# Autodesk Inventor assembly: GripCharger
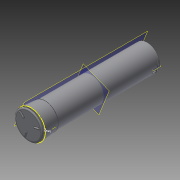
[picture p0: Inventor's stored thumbnail of the model, 180x180]
Saved by Autodesk Inventor 2014 SP1 (Build 180222100, 222)
## iProperties
Created: 2015-10-17
Part Number: GripCharger
Document SubType Name: Assembly
Designer: anthony
Author: anthony
## Documents named in this file (4)
- C:\Users\anthony\Documents\HardwareHack\GripCharger.iam
- C:\Users\anthony\Documents\HardwareHack\GripOuterTube.ipt
- C:\Users\anthony\Documents\HardwareHack\GripScrewCap.ipt
- C:\Users\anthony\Documents\HardwareHack\GripScrewCapCap.ipt
## Components (3 placed, 3 different names)
1. GripOuterTube:1 — Mate:1, Mate:2, Mate:3
2. GripScrewCap:1 — Mate:1, Mate:3
3. GripScrewCapCap:1
## Relationships (3: Mate 3)
- Mate:1: GripOuterTube:1 ↔ GripScrewCap:1
- Mate:2: GripOuterTube:1
- Mate:3: GripOuterTube:1 ↔ GripScrewCap:1
